# Autodesk Inventor assembly: hood prototype
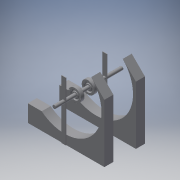
[picture p0: Inventor's stored thumbnail of the model, 180x180]
Saved by Autodesk Inventor 2018 (Build 220112000, 112)
## iProperties
Created: 2020-01-10
Part Number: hood prototype
Document SubType Name: Assembly
Designer: s-2513225
Author: s-2513225
## Documents named in this file (5)
- \\studenthome\students\S-2513225\ROBOTICS\2020\Hood outtake 3d print part\hood prototype.iam
- \\studenthome\students\S-2513225\ROBOTICS\2020\Hood outtake 3d print part\main prototype.ipt
- \\studenthome\students\S-2513225\ROBOTICS\2020\T81P-29.ipt
- \\studenthome\students\S-2513225\ROBOTICS\2020\Hood outtake 3d print part\wall.ipt
- \\studenthome\students\S-2513225\ROBOTICS\2020\Hood outtake 3d print part\rod.ipt
## Components (7 placed, 4 different names)
1. main prototype:1 — Flush:2, Mate:2, Flush:3, Flush:4, Mate:7
2. main prototype:2 — Mate:1, Flush:1, Flush:3, Flush:4, Mate:5, Mate:6, Mate:8
3. T81P-29:1 — Mate:4
4. T81P-29:2 — Mate:3
5. wall:1 — Mate:1, Flush:1, Mate:3, Flush:5, Mate:9
6. wall:2 — Flush:2, Mate:2, Mate:4, Flush:5
7. rod:1 — Mate:9
## Relationships (14: Mate 9, Flush 5)
- Mate:1: main prototype:2 ↔ wall:1
- Flush:1: main prototype:2 ↔ wall:1
- Flush:2: main prototype:1 ↔ wall:2
- Mate:2: main prototype:1 ↔ wall:2
- Flush:3: main prototype:1 ↔ main prototype:2
- Flush:4: main prototype:1 ↔ main prototype:2
- Mate:3: T81P-29:2 ↔ wall:1
- Mate:4: T81P-29:1 ↔ wall:2
- Flush:5: wall:1 ↔ wall:2
- Mate:5: main prototype:2
- Mate:6 (-88.9 mm): main prototype:2
- Mate:7 (88.9 mm): main prototype:1
- Mate:8: main prototype:2
- Mate:9: wall:1 ↔ rod:1
